# Autodesk Inventor assembly: case
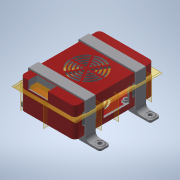
[picture p0: Inventor's stored thumbnail of the model, 180x180]
Saved by Autodesk Inventor 2020 (Build 240168000, 168)
## iProperties
Created: 2019-03-26
Part Number: case
Document SubType Name: Assembly
Designer: erwin
Author: erwin
## Documents named in this file (4)
- D:\GitHub\ElCheapoAIS-nmea\case\source\case.iam
- D:\GitHub\ElCheapoAIS-nmea\case\source\top_part.ipt
- D:\GitHub\ElCheapoAIS-nmea\case\source\bottom_part.ipt
- D:\GitHub\ElCheapoAIS-nmea\case\source\rail_clip_branded.ipt
## Components (4 placed, 3 different names)
1. top_part:1 — Mate:1, Mate:4
2. bottom_part:1 — Mate:2, Mate:3
3. rail_clip_branded:1 — Mate:1, Mate:2
4. rail_clip_branded:2 — Mate:3, Mate:4
## Relationships (4: Mate 4)
- Mate:1: top_part:1 ↔ rail_clip_branded:1
- Mate:2: bottom_part:1 ↔ rail_clip_branded:1
- Mate:3: bottom_part:1 ↔ rail_clip_branded:2
- Mate:4: top_part:1 ↔ rail_clip_branded:2
